# Autodesk Inventor assembly: mascon-new
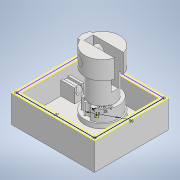
[picture p0: Inventor's stored thumbnail of the model, 180x180]
Saved by Autodesk Inventor 2021 (Build 250183000, 183)
## iProperties
Created: 2021-04-28
Part Number: mascon-new
Document SubType Name: Assembly
Designer: ben
Author: ben
## Documents named in this file (6)
- C:\Users\teh18\OneDrive\BVE Controller\r68-bve-mascon\mascon-new.iam
- C:\Users\teh18\OneDrive\BVE Controller\r68-bve-mascon\mascon.ipt
- C:\Users\teh18\OneDrive\BVE Controller\r68-bve-mascon\handle_base.ipt
- C:\Users\teh18\OneDrive\BVE Controller\r68-bve-mascon\handle_base2.ipt
- C:\Users\teh18\OneDrive\BVE Controller\r68-bve-mascon\stl2\HandleRod1.ipt
- C:\Users\teh18\OneDrive\BVE Controller\r68-bve-mascon\stl2\NotchPiston1.ipt
## Components (5 placed, 5 different names)
1. mascon:1 — Flush:3
2. handle_base:1 — Flush:1, Flush:2
3. handle_base2:1 — Flush:1
4. HandleRod1:1 — Flush:2
5. NotchPiston1:1 — Flush:3
## Relationships (3: Flush 3)
- Flush:1: handle_base:1 ↔ handle_base2:1
- Flush:2: handle_base:1 ↔ HandleRod1:1
- Flush:3: mascon:1 ↔ NotchPiston1:1
